# Autodesk Inventor assembly: ModuloExtractor
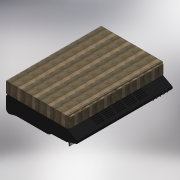
[picture p0: Inventor's stored thumbnail of the model, 180x180]
Saved by Autodesk Inventor 2016 (Build 200138000, 138)
## iProperties
Created: 2015-11-24
Part Number: ModuloExtractor
Material: Genérico
Document SubType Name: Assembly
Designer: eolun
Author: eolun
## Documents named in this file (4)
- C:\Users\Sebastian\Desktop\sebas\trabajos\COCINA FINAAAAAAAAAAAL\COCINA FINAAAAAAAAAAAL\Cocina\Cocina\ModuloExtractor.iam
- C:\Users\Sebastian\Desktop\sebas\trabajos\COCINA FINAAAAAAAAAAAL\COCINA FINAAAAAAAAAAAL\Cocina\Cocina\Extractor.ipt
- C:\Users\Sebastian\Desktop\sebas\trabajos\COCINA FINAAAAAAAAAAAL\COCINA FINAAAAAAAAAAAL\Cocina\Cocina\MuebleExtractor.ipt
- C:\Users\Sebastian\Desktop\sebas\trabajos\COCINA FINAAAAAAAAAAAL\COCINA FINAAAAAAAAAAAL\Cocina\Cocina\manija.ipt
## Components (4 placed, 3 different names)
1. Extractor:1 — Coincidencia:1, Nivelación:1, Coincidencia:2
2. MuebleExtractor:1 — Coincidencia:1, Nivelación:1, Coincidencia:2, Coincidencia:3, Coincidencia:4, Coincidencia:5, Coincidencia:6, Coincidencia:7, Coincidencia:8
3. manija:1 — Coincidencia:3, Coincidencia:4, Coincidencia:5
4. manija:2 — Coincidencia:6, Coincidencia:7, Coincidencia:8
## Relationships (9: Mate 8, Flush 1)
- Coincidencia:1 [Mate]: Extractor:1 ↔ MuebleExtractor:1
- Nivelación:1 [Flush]: Extractor:1 ↔ MuebleExtractor:1
- Coincidencia:2 [Mate]: Extractor:1 ↔ MuebleExtractor:1
- Coincidencia:3 [Mate]: MuebleExtractor:1 ↔ manija:1
- Coincidencia:4 [Mate]: MuebleExtractor:1 ↔ manija:1
- Coincidencia:5 [Mate]: MuebleExtractor:1 ↔ manija:1
- Coincidencia:6 [Mate]: MuebleExtractor:1 ↔ manija:2
- Coincidencia:7 [Mate]: MuebleExtractor:1 ↔ manija:2
- Coincidencia:8 [Mate]: MuebleExtractor:1 ↔ manija:2
